# Autodesk Inventor assembly: main
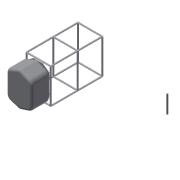
[picture p0: Inventor's stored thumbnail of the model, 180x180]
Saved by Autodesk Inventor 2014 SP1 (Build 180222100, 222)
## iProperties
Created: 2015-02-04
Part Number: main
Document SubType Name: Assembly
Designer: Simen
Author: Simen
## Documents named in this file (4)
- C:\Users\Simen\Documents\git\Eit\skjellet\main.iam
- C:\Users\Simen\Documents\git\Eit\skjellet\base.iam
- C:\Users\Simen\Documents\git\Eit\skjellet\skellett.iam
- C:\Users\Simen\Documents\git\Eit\skjellet\KHFS5_2020_350.ipt
## Components (3 placed, 3 different names)
1. base:1 [sub-assembly] — Mate:1, Flush:1
2. skellett:1 [sub-assembly] — Mate:1, Flush:1
3. KHFS5-2020-4000:1
## Relationships (2: Mate 1, Flush 1)
- Mate:1: base:1 ↔ skellett:1
- Flush:1: base:1 ↔ skellett:1
